# Autodesk Inventor assembly: robot
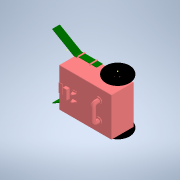
[picture p0: Inventor's stored thumbnail of the model, 180x180]
Saved by Autodesk Inventor 2020 (Build 240168000, 168)
## iProperties
Created: 2023-01-13
Part Number: robot
Document SubType Name: Assembly
Designer: hugoG
Author: hugoG
## Documents named in this file (9)
- D:\cours ensta\3A\IG\robot.iam
- D:\cours ensta\3A\IG\corps.ipt
- D:\cours ensta\3A\IG\wheel.ipt
- D:\cours ensta\3A\IG\support pelle.ipt
- D:\cours ensta\3A\IG\Assembly2.iam
- D:\cours ensta\3A\IG\ramasse r.ipt
- D:\cours ensta\3A\IG\fixation ramasse.ipt
- D:\cours ensta\3A\IG\ramasse l.ipt
- D:\cours ensta\3A\IG\poignet.ipt
## Components (14 placed, 8 different names)
1. corps:1 — Mate:1, Mate:2, Mate:3, Mate:4, Mate:11, Mate:12, Mate:13, Mate:14, Mate:15, Mate:16, Mate:20, Mate:21, Mate:22, Mate:23, Mate:24, Mate:25, Mate:26, Mate:27, Mate:28, Mate:29, Mate:30, Mate:33, Mate:34, Mate:35, Mate:36, Mate:37, Mate:38, Mate:39, Mate:42, Mate:43, Mate:44
2. wheel:1 — Mate:1, Mate:2
3. wheel:2 — Mate:3, Mate:4
4. support pelle:1 — Mate:12, Mate:15, Mate:16
5. support pelle:2 — Mate:11, Mate:13, Mate:14
6. Assembly2:1 [sub-assembly] — Mate:21, Mate:24, Mate:25
7. Assembly2:2 [sub-assembly] — Mate:20, Mate:22, Mate:23
8. ramasse r:1 — Mate:39, Mate:40, Mate:41
9. fixation ramasse:1 — Mate:28, Mate:29
10. fixation ramasse:2 — Mate:26, Mate:27, Mate:31, Mate:32
11. fixation ramasse:3 — Mate:36, Mate:37, Mate:38
12. fixation ramasse:4 — Mate:33, Mate:34, Mate:35, Mate:40, Mate:41
13. ramasse l:1 — Mate:30, Mate:31, Mate:32
14. poignet:1 — Mate:42, Mate:43, Mate:44
## Relationships (35: Mate 35)
- Mate:1: corps:1 ↔ wheel:1
- Mate:2: corps:1 ↔ wheel:1
- Mate:3: corps:1 ↔ wheel:2
- Mate:4: corps:1 ↔ wheel:2
- Mate:11: corps:1 ↔ support pelle:2
- Mate:12: corps:1 ↔ support pelle:1
- Mate:13: corps:1 ↔ support pelle:2
- Mate:14: corps:1 ↔ support pelle:2
- Mate:15: corps:1 ↔ support pelle:1
- Mate:16: corps:1 ↔ support pelle:1
- Mate:20: corps:1 ↔ Assembly2:2
- Mate:21: corps:1 ↔ Assembly2:1
- Mate:22: corps:1 ↔ Assembly2:2
- Mate:23: corps:1 ↔ Assembly2:2
- Mate:24: corps:1 ↔ Assembly2:1
- Mate:25: corps:1 ↔ Assembly2:1
- Mate:26: corps:1 ↔ fixation ramasse:2
- Mate:27: corps:1 ↔ fixation ramasse:2
- Mate:28: corps:1 ↔ fixation ramasse:1
- Mate:29: corps:1 ↔ fixation ramasse:1
- Mate:30: corps:1 ↔ ramasse l:1
- Mate:31: fixation ramasse:2 ↔ ramasse l:1
- Mate:32: fixation ramasse:2 ↔ ramasse l:1
- Mate:33: corps:1 ↔ fixation ramasse:4
- Mate:34: corps:1 ↔ fixation ramasse:4
- Mate:35: corps:1 ↔ fixation ramasse:4
- Mate:36: corps:1 ↔ fixation ramasse:3
- Mate:37: corps:1 ↔ fixation ramasse:3
- Mate:38: corps:1 ↔ fixation ramasse:3
- Mate:39: corps:1 ↔ ramasse r:1
- Mate:40: ramasse r:1 ↔ fixation ramasse:4
- Mate:41: ramasse r:1 ↔ fixation ramasse:4
- Mate:42: corps:1 ↔ poignet:1
- Mate:43: corps:1 ↔ poignet:1
- Mate:44: corps:1 ↔ poignet:1
